# Autodesk Inventor assembly: 01-3
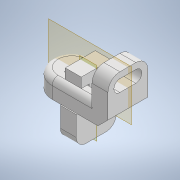
[picture p0: Inventor's stored thumbnail of the model, 180x180]
Saved by Autodesk Inventor 2022 (Build 260153000, 153)
## iProperties
Created: 2021-09-11
Part Number: 01-3
Document SubType Name: Assembly
Designer: 서울공업고등학교
Author: 서울공업고등학교
## Documents named in this file (3)
- C:\Users\서울공업고등학교\Documents\_9_11\01-3.iam
- C:\Users\서울공업고등학교\Documents\_9_11\모의고사1\1번부품.ipt
- C:\Users\서울공업고등학교\Downloads\aa\3dPrinter-main\_9_4\모의고사1\2번부품.ipt
## Components (2 placed, 2 different names)
1. 1번부품:1 — 메이트:1, 메이트:2
2. 2번부품:1 — 메이트:1, 메이트:2
## Relationships (2: Mate 2)
- 메이트:1 [Mate]: 1번부품:1 ↔ 2번부품:1
- 메이트:2 [Mate] (0.5 mm): 1번부품:1 ↔ 2번부품:1
